# Autodesk Inventor assembly: main
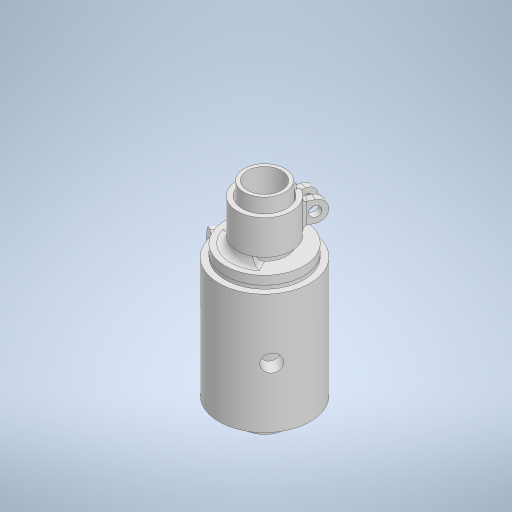
[picture p0: Inventor's stored thumbnail of the model, 512x512]
Saved by Autodesk Inventor 2023 (Build 270158000, 158)
## iProperties
Created: 2024-07-20
Part Number: main
Document SubType Name: Assembly
Designer: plebbb
Author: plebbb
## Documents named in this file (5)
- C:\Users\plebbb\Desktop\Dial_indicator_mount\main.iam
- C:\Users\plebbb\Desktop\Dial_indicator_mount\6703ZZ.ipt
- C:\Users\plebbb\Desktop\Dial_indicator_mount\External_roller.ipt
- C:\Users\plebbb\Desktop\Dial_indicator_mount\12mm_shaft.ipt
- C:\Users\plebbb\Desktop\Dial_indicator_mount\Internal_roller.ipt
## Components (5 placed, 4 different names)
1. 6703ZZ:1 — Mate:6, Mate:7
2. External_roller:1 — Mate:4, Mate:5, Mate:6
3. 6703ZZ:2 — Mate:2, Mate:3, Mate:4
4. 12mm_shaft:1 — Mate:1
5. Internal_roller:1 — Mate:1, Mate:2, Mate:3, Mate:5, Mate:7
## Relationships (7: Mate 7)
- Mate:1: 12mm_shaft:1 ↔ Internal_roller:1
- Mate:2: 6703ZZ:2 ↔ Internal_roller:1
- Mate:3: 6703ZZ:2 ↔ Internal_roller:1
- Mate:4: External_roller:1 ↔ 6703ZZ:2
- Mate:5: External_roller:1 ↔ Internal_roller:1
- Mate:6: 6703ZZ:1 ↔ External_roller:1
- Mate:7: 6703ZZ:1 ↔ Internal_roller:1
